# Autodesk Inventor assembly: RedHP
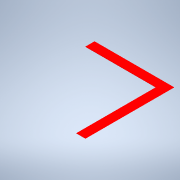
[picture p0: Inventor's stored thumbnail of the model, 180x180]
Saved by Autodesk Inventor 2021 (Build 250183000, 183)
## iProperties
Created: 2021-03-04
Part Number: RedHP
Document SubType Name: Assembly
Designer: CMurray
Author: CMurray
## Documents named in this file (2)
- F:\PHRC CADD 2021\2021 Game Design Challenge\Full Field\Parts\Tape\RedHP.iam
- F:\PHRC CADD 2021\2021 Game Design Challenge\Full Field\Parts\Tape\BlueAllianceTape-ver1-1111-2021.ipt
## Components (2 placed, 1 different names)
1. BlueAllianceTape-ver1-1111-2021:1 — Flush:1, Mate:1, Flush:2
2. BlueAllianceTape-ver1-1111-2021:2 — Flush:1, Mate:1, Flush:2
## Relationships (3: Flush 2, Mate 1)
- Flush:1: BlueAllianceTape-ver1-1111-2021:1 ↔ BlueAllianceTape-ver1-1111-2021:2
- Mate:1: BlueAllianceTape-ver1-1111-2021:1 ↔ BlueAllianceTape-ver1-1111-2021:2
- Flush:2: BlueAllianceTape-ver1-1111-2021:1 ↔ BlueAllianceTape-ver1-1111-2021:2
